# Autodesk Inventor assembly: Elo_sup
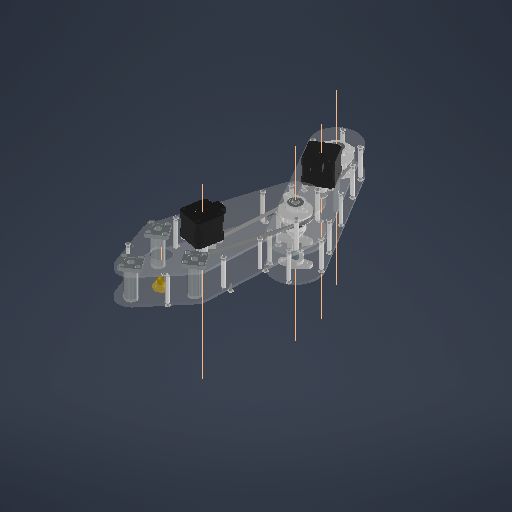
[picture p0: Inventor's stored thumbnail of the model, 512x512]
Saved by Autodesk Inventor 2025.2 (Build 292293000, 293)
## iProperties
Created: 2025-04-19
Part Number: Elo_sup
Document SubType Name: Assembly
Designer: Nelson
Author: Nelson
## Documents named in this file (19)
- C:\Users\Tiago\Documents\Inventor\Exp. Braço v1\Elo_sup.iam
- C:\Users\Tiago\Documents\Inventor\Exp. Braço v1\Veio_D8mm_L100mm.ipt
- C:\Users\Tiago\Documents\Inventor\Exp. Braço v1\RolamentoLinear10d.ipt
- C:\Users\Tiago\Documents\Inventor\Exp. Braço v1\KFL08 - Mancal Flange oval Ø8.ipt
- C:\Users\Tiago\Documents\Inventor\Exp. Braço v1\NEMA17 42-38.ipt
- C:\Users\Tiago\Documents\Inventor\Exp. Braço v1\Porca_T8.ipt
- C:\Users\Tiago\Documents\Inventor\Exp. Braço v1\Linear_Shaft_Support_SHF8.ipt
- C:\Users\Tiago\Documents\Inventor\Exp. Braço v1\1ELO.ipt
- C:\Users\Tiago\Documents\Inventor\Exp. Braço v1\2ELO.ipt
- C:\Users\Tiago\Documents\Inventor\Exp. Braço v1\3ELO.ipt
- C:\Users\Tiago\Documents\Inventor\Exp. Braço v1\4ELO.ipt
- C:\Users\Tiago\Documents\Inventor\Exp. Braço v1\espaçador_M3_L40.ipt
- C:\Users\Tiago\Documents\Inventor\Exp. Braço v1\GT2Pulley_z60.ipt
- C:\Users\Tiago\Documents\Inventor\Exp. Braço v1\GT2Pulley_z20.ipt
- C:\Users\Tiago\Documents\Inventor\Exp. Braço v1\Elo_sup\Design Accelerator\Synchronous Belts Transmission3.iam
- C:\Users\Tiago\Documents\Inventor\Exp. Braço v1\Limit_Switch_L1.ipt
- C:\Users\Tiago\Documents\Inventor\Exp. Braço v1\Elo_sup\Design Accelerator\Synchronous Belts Transmission5.iam
- C:\Users\Tiago\Documents\Inventor\Exp. Braço v1\M3 x0.5 ALT (...).ipt
- C:\Users\Tiago\Documents\Inventor\Exp. Braço v1\Anilha_M3.ipt
## Components (146 placed, 17 different names)
1. Veio_D8mm_L100mm:1 — Mate:45, Mate:48, Mate:61, Flush:3, Mate:64, Mate:65, Mate:78, Mate:82, Flush:5, Mate:143, Rotation:3, Rotation:4
2. RolamentoLinear10d:1 — Mate:54, Mate:68, Flush:4, Mate:192, Mate:193
3. RolamentoLinear10d:2 — Mate:56, Mate:190, Mate:191
4. RolamentoLinear10d:3 — Mate:57, Mate:70, Mate:194, Mate:195
5. KFL08 - Mancal Flange oval Ø8:1 — Mate:65, Mate:71, Mate:91
6. KFL08 - Mancal Flange oval Ø8:2 — Mate:63, Mate:64, Mate:74, Mate:75
7. NEMA17 42-38:1 — Mate:98, Mate:141, Mate:144, Flush:161
8. Porca_T8:1 — Mate:66, Mate:67, Mate:76, Mate:77
9. NEMA17 42-38:2 — Mate:162, Mate:163, Mate:164, Flush:159
10. Linear_Shaft_Support_SHF8:1 — Mate:45, Mate:80, Mate:81
11. Linear_Shaft_Support_SHF8:2 — Mate:48, Mate:83, Mate:84
12. Veio_D8mm_L100mm:2 — Mate:51, Mate:53, Mate:85, Mate:86, Flush:6, Mate:149
13. KFL08 - Mancal Flange oval Ø8:3 — Mate:51, Mate:87, Mate:88
14. KFL08 - Mancal Flange oval Ø8:4 — Mate:53, Mate:89, Mate:90
15. 1ELO:1 — Mate:54, Mate:56, Mate:57, Mate:61, Flush:3, Mate:63, Mate:74, Mate:75, Mate:98, Mate:100, Mate:101, Mate:102, Mate:103, Mate:104, Mate:105, Mate:106, Mate:107, Mate:121, Mate:127, Mate:144, Mate:145, Mate:146, Flush:158, Mate:157, Insert:1, Insert:4, Insert:6, Insert:8, Insert:10, Insert:12, Insert:14, Insert:16, Insert:18, Mate:182, Mate:183, Mate:184, Mate:185, Mate:186, Mate:187, Mate:188, Mate:189, Mate:190, Mate:191, Mate:192, Mate:193, Mate:194, Mate:195
16. 2ELO:1 — Mate:66, Mate:67, Mate:68, Mate:70, Flush:4, Mate:71, Mate:76, Mate:77, Distância dos elos, Mate:91, Mate:99, Mate:120, Mate:122, Mate:123, Mate:124, Mate:125, Mate:126, Mate:128, Mate:159, Mate:160, Mate:161, Angle:1, Insert:28, Insert:30, Insert:32, Insert:74, Insert:78, Insert:80, Insert:82, Insert:84, Flush:161, Insert:93
17. 3ELO:1 — Mate:78, Distância dos elos, Mate:80, Mate:81, Mate:85, Flush:6, Mate:87, Mate:88, Mate:129, Mate:130, Mate:131, Mate:132, Mate:133, Mate:134, Mate:135, Mate:136, Mate:137, Mate:138, Mate:139, Mate:140, Rotation:4, Mate:162, Mate:163, Mate:166, Mate:173, Insert:20, Insert:22, Insert:24, Insert:26, Insert:34, Insert:36, Insert:38, Insert:40, Insert:42, Insert:44, Insert:46, Insert:48, Mate:174, Mate:175, Mate:176, Mate:177, Mate:178, Mate:179, Mate:180, Mate:181
18. 4ELO:1 — Mate:82, Flush:5, Mate:83, Mate:84, Mate:86, Mate:89, Mate:90, Mate:108, Mate:109, Mate:110, Mate:111, Mate:112, Mate:113, Mate:114, Mate:115, Mate:116, Mate:117, Mate:118, Mate:119, Angle:1, Mate:167, Flush:159, Mate:173, Insert:50, Insert:52, Insert:54, Insert:56, Insert:58, Insert:60, Insert:62, Insert:64, Insert:66, Insert:68, Insert:70, Insert:94
19. espaçador_M3_L40:1 — Mate:99, Mate:100
20. espaçador_M3_L40:2 — Mate:101, Mate:126
21. espaçador_M3_L40:3 — Mate:103, Mate:123
22. espaçador_M3_L40:4 — Mate:105, Mate:122
23. espaçador_M3_L40:5 — Mate:102, Mate:127
24. espaçador_M3_L40:6 — Mate:107, Mate:125
25. espaçador_M3_L40:7 — Mate:108, Mate:130
26. espaçador_M3_L40:8 — Mate:109, Mate:131
27. espaçador_M3_L40:9 — Mate:104, Mate:128
28. espaçador_M3_L40:10 — Mate:106, Mate:124
29. espaçador_M3_L40:11 — Mate:110, Mate:129
30. espaçador_M3_L40:12 — Mate:111, Mate:135
31. espaçador_M3_L40:13 — Mate:114, Mate:138
32. espaçador_M3_L40:14 — Mate:113, Mate:139
33. espaçador_M3_L40:15 — Mate:112, Mate:140
34. espaçador_M3_L40:16 — Mate:115, Mate:136
35. espaçador_M3_L40:17 — Mate:116, Mate:137
36. espaçador_M3_L40:18 — Mate:117, Mate:134
37. espaçador_M3_L40:20 — Mate:119, Mate:132
38. espaçador_M3_L40:21 — Mate:120, Mate:121
39. espaçador_M3_L40:22 — Mate:118, Mate:133
40. GT2Pulley_z60:1 — Mate:143, Mate:145, Mate:148, Flush:7, Rotation:1, Rotation:3
41. GT2Pulley_z20:1 — Mate:141, Mate:146, Mate:147, Rotation:1
42. Synchronous Belts Transmission:3 [sub-assembly] — Mate:147, Mate:148, Flush:7
43. GT2Pulley_z20:2 — Rotation:2, Mate:164, Mate:167, Mate:169
44. GT2Pulley_z60:2 — Mate:149, Rotation:2, Mate:166, Mate:168, Flush:160
45. Limit_Switch_L1:1 — Mate:159, Mate:160, Mate:161
46. Synchronous Belts Transmission:4 [sub-assembly] — Mate:168, Mate:169, Flush:160
47. M3 x0.5 ALT (...):1 — Insert:2
48. Anilha_M3:1 — Insert:1, Insert:2
49. M3 x0.5 ALT (...):2
50. Anilha_M3:2 — Insert:4
51. M3 x0.5 ALT (...):3
52. Anilha_M3:3 — Insert:6
53. M3 x0.5 ALT (...):4
54. Anilha_M3:4 — Insert:8
55. M3 x0.5 ALT (...):5
56. Anilha_M3:5 — Insert:10
57. M3 x0.5 ALT (...):6
58. Anilha_M3:6 — Insert:12
59. M3 x0.5 ALT (...):7
60. Anilha_M3:7 — Insert:14
61. M3 x0.5 ALT (...):8
62. Anilha_M3:8 — Insert:16
63. M3 x0.5 ALT (...):9
64. Anilha_M3:9 — Insert:18
65. M3 x0.5 ALT (...):10
66. Anilha_M3:10 — Insert:20
67. M3 x0.5 ALT (...):11
68. Anilha_M3:11 — Insert:22
69. M3 x0.5 ALT (...):12
70. Anilha_M3:12 — Insert:24
71. M3 x0.5 ALT (...):13
72. Anilha_M3:13 — Insert:26
73. M3 x0.5 ALT (...):14
74. Anilha_M3:14 — Insert:28
75. M3 x0.5 ALT (...):15
76. Anilha_M3:15 — Insert:30
77. M3 x0.5 ALT (...):16
78. Anilha_M3:16 — Insert:32
79. M3 x0.5 ALT (...):17
80. Anilha_M3:17 — Insert:34
81. M3 x0.5 ALT (...):18
82. Anilha_M3:18 — Insert:36
83. M3 x0.5 ALT (...):19
84. Anilha_M3:19 — Insert:38
85. M3 x0.5 ALT (...):20
86. Anilha_M3:20 — Insert:40
87. M3 x0.5 ALT (...):21
88. Anilha_M3:21 — Insert:42
89. M3 x0.5 ALT (...):22
90. Anilha_M3:22 — Insert:44
91. M3 x0.5 ALT (...):23
92. Anilha_M3:23 — Insert:46
93. M3 x0.5 ALT (...):24
94. Anilha_M3:24 — Insert:48
95. M3 x0.5 ALT (...):25
96. Anilha_M3:25 — Insert:50
97. M3 x0.5 ALT (...):26
98. Anilha_M3:26 — Insert:52
99. M3 x0.5 ALT (...):27
100. Anilha_M3:27 — Insert:54
101. M3 x0.5 ALT (...):28
102. Anilha_M3:28 — Insert:56
103. M3 x0.5 ALT (...):29
104. Anilha_M3:29 — Insert:58
105. M3 x0.5 ALT (...):30
106. Anilha_M3:30 — Insert:60
107. M3 x0.5 ALT (...):31
108. Anilha_M3:31 — Insert:62
109. M3 x0.5 ALT (...):32
110. Anilha_M3:32 — Insert:64
111. M3 x0.5 ALT (...):33
112. Anilha_M3:33 — Insert:66
113. M3 x0.5 ALT (...):34
114. Anilha_M3:34 — Insert:68
115. M3 x0.5 ALT (...):35
116. Anilha_M3:35 — Insert:70
117. M3 x0.5 ALT (...):36
118. Anilha_M3:36 — Insert:94
119. M3 x0.5 ALT (...):37
120. Anilha_M3:37 — Insert:74
121. M3 x0.5 ALT (...):38
122. Anilha_M3:38 — Insert:93
123. M3 x0.5 ALT (...):39
124. Anilha_M3:39 — Insert:78
125. M3 x0.5 ALT (...):40
126. Anilha_M3:40 — Insert:80
127. M3 x0.5 ALT (...):41
128. Anilha_M3:41 — Insert:82
129. M3 x0.5 ALT (...):42
130. Anilha_M3:42 — Insert:84
131. M3 x0.5 ALT (...):43 — Mate:174
132. Anilha_M3:43 — Mate:175
133. M3 x0.5 ALT (...):44 — Mate:176
134. Anilha_M3:44 — Mate:177
135. M3 x0.5 ALT (...):45 — Mate:178
136. Anilha_M3:45 — Mate:181
137. M3 x0.5 ALT (...):46 — Mate:179
138. Anilha_M3:46 — Mate:180
139. M3 x0.5 ALT (...):47 — Mate:182
140. Anilha_M3:47 — Mate:187
141. M3 x0.5 ALT (...):48 — Mate:183
142. Anilha_M3:48 — Mate:189
143. M3 x0.5 ALT (...):49 — Mate:184
144. Anilha_M3:49 — Mate:186
145. M3 x0.5 ALT (...):50 — Mate:185
146. Anilha_M3:50 — Mate:188
## Relationships (226: Mate 119, Insert 92, Flush 10, RelateRotation 4, Angle 1)
- Flush:2 (-10 mm)
- Mate:45: Veio_D8mm_L100mm:1 ↔ Linear_Shaft_Support_SHF8:1
- Mate:48: Veio_D8mm_L100mm:1 ↔ Linear_Shaft_Support_SHF8:2
- Mate:51: Veio_D8mm_L100mm:2 ↔ KFL08 - Mancal Flange oval Ø8:3
- Mate:53: Veio_D8mm_L100mm:2 ↔ KFL08 - Mancal Flange oval Ø8:4
- Mate:54: RolamentoLinear10d:1 ↔ 1ELO:1
- Mate:56: RolamentoLinear10d:2 ↔ 1ELO:1
- Mate:57: RolamentoLinear10d:3 ↔ 1ELO:1
- Mate:61: Veio_D8mm_L100mm:1 ↔ 1ELO:1
- Flush:3 (-1 mm): Veio_D8mm_L100mm:1 ↔ 1ELO:1
- Mate:63: KFL08 - Mancal Flange oval Ø8:2 ↔ 1ELO:1
- Mate:64: Veio_D8mm_L100mm:1 ↔ KFL08 - Mancal Flange oval Ø8:2
- Mate:65: Veio_D8mm_L100mm:1 ↔ KFL08 - Mancal Flange oval Ø8:1
- Mate:66: Porca_T8:1 ↔ 2ELO:1
- Mate:67: Porca_T8:1 ↔ 2ELO:1
- Mate:68: RolamentoLinear10d:1 ↔ 2ELO:1
- Mate:70: RolamentoLinear10d:3 ↔ 2ELO:1
- Flush:4 (-1 mm): RolamentoLinear10d:1 ↔ 2ELO:1
- Mate:71: KFL08 - Mancal Flange oval Ø8:1 ↔ 2ELO:1
- Mate:74: KFL08 - Mancal Flange oval Ø8:2 ↔ 1ELO:1
- Mate:75: KFL08 - Mancal Flange oval Ø8:2 ↔ 1ELO:1
- Mate:76: Porca_T8:1 ↔ 2ELO:1
- Mate:77: Porca_T8:1 ↔ 2ELO:1
- Mate:78: Veio_D8mm_L100mm:1 ↔ 3ELO:1
- Distância dos elos [Mate] (6 mm): 2ELO:1 ↔ 3ELO:1
- Mate:80: Linear_Shaft_Support_SHF8:1 ↔ 3ELO:1
- Mate:81: Linear_Shaft_Support_SHF8:1 ↔ 3ELO:1
- Mate:82: Veio_D8mm_L100mm:1 ↔ 4ELO:1
- Flush:5: Veio_D8mm_L100mm:1 ↔ 4ELO:1
- Mate:83: Linear_Shaft_Support_SHF8:2 ↔ 4ELO:1
- Mate:84: Linear_Shaft_Support_SHF8:2 ↔ 4ELO:1
- Mate:85: Veio_D8mm_L100mm:2 ↔ 3ELO:1
- Mate:86: Veio_D8mm_L100mm:2 ↔ 4ELO:1
- Flush:6: Veio_D8mm_L100mm:2 ↔ 3ELO:1
- Mate:87: KFL08 - Mancal Flange oval Ø8:3 ↔ 3ELO:1
- Mate:88: KFL08 - Mancal Flange oval Ø8:3 ↔ 3ELO:1
- Mate:89: KFL08 - Mancal Flange oval Ø8:4 ↔ 4ELO:1
- Mate:90: KFL08 - Mancal Flange oval Ø8:4 ↔ 4ELO:1
- Mate:91: KFL08 - Mancal Flange oval Ø8:1 ↔ 2ELO:1
- Mate:98: NEMA17 42-38:1 ↔ 1ELO:1
- Mate:99: 2ELO:1 ↔ espaçador_M3_L40:1
- Mate:100: 1ELO:1 ↔ espaçador_M3_L40:1
- Mate:101: 1ELO:1 ↔ espaçador_M3_L40:2
- Mate:102: 1ELO:1 ↔ espaçador_M3_L40:5
- Mate:103: 1ELO:1 ↔ espaçador_M3_L40:3
- Mate:104: 1ELO:1 ↔ espaçador_M3_L40:9
- Mate:105: 1ELO:1 ↔ espaçador_M3_L40:4
- Mate:106: 1ELO:1 ↔ espaçador_M3_L40:10
- Mate:107: 1ELO:1 ↔ espaçador_M3_L40:6
- Mate:108: 4ELO:1 ↔ espaçador_M3_L40:7
- Mate:109: 4ELO:1 ↔ espaçador_M3_L40:8
- Mate:110: 4ELO:1 ↔ espaçador_M3_L40:11
- Mate:111: 4ELO:1 ↔ espaçador_M3_L40:12
- Mate:112: 4ELO:1 ↔ espaçador_M3_L40:15
- Mate:113: 4ELO:1 ↔ espaçador_M3_L40:14
- Mate:114: 4ELO:1 ↔ espaçador_M3_L40:13
- Mate:115: 4ELO:1 ↔ espaçador_M3_L40:16
- Mate:116: 4ELO:1 ↔ espaçador_M3_L40:17
- Mate:117: 4ELO:1 ↔ espaçador_M3_L40:18
- Mate:118: 4ELO:1 ↔ espaçador_M3_L40:22
- Mate:119: 4ELO:1 ↔ espaçador_M3_L40:20
- Mate:120: 2ELO:1 ↔ espaçador_M3_L40:21
- Mate:121: 1ELO:1 ↔ espaçador_M3_L40:21
- Mate:122: 2ELO:1 ↔ espaçador_M3_L40:4
- Mate:123: 2ELO:1 ↔ espaçador_M3_L40:3
- Mate:124: 2ELO:1 ↔ espaçador_M3_L40:10
- Mate:125: 2ELO:1 ↔ espaçador_M3_L40:6
- Mate:126: 2ELO:1 ↔ espaçador_M3_L40:2
- Mate:127: 1ELO:1 ↔ espaçador_M3_L40:5
- Mate:128: 2ELO:1 ↔ espaçador_M3_L40:9
- Mate:129: 3ELO:1 ↔ espaçador_M3_L40:11
- Mate:130: 3ELO:1 ↔ espaçador_M3_L40:7
- Mate:131: 3ELO:1 ↔ espaçador_M3_L40:8
- Mate:132: 3ELO:1 ↔ espaçador_M3_L40:20
- Mate:133: 3ELO:1 ↔ espaçador_M3_L40:22
- Mate:134: 3ELO:1 ↔ espaçador_M3_L40:18
- Mate:135: 3ELO:1 ↔ espaçador_M3_L40:12
- Mate:136: 3ELO:1 ↔ espaçador_M3_L40:16
- Mate:137: 3ELO:1 ↔ espaçador_M3_L40:17
- Mate:138: 3ELO:1 ↔ espaçador_M3_L40:13
- Mate:139: 3ELO:1 ↔ espaçador_M3_L40:14
- Mate:140: 3ELO:1 ↔ espaçador_M3_L40:15
- Mate:141: NEMA17 42-38:1 ↔ GT2Pulley_z20:1
- Mate:143: Veio_D8mm_L100mm:1 ↔ GT2Pulley_z60:1
- Mate:144: NEMA17 42-38:1 ↔ 1ELO:1
- Mate:145 (12 mm): 1ELO:1 ↔ GT2Pulley_z60:1
- Mate:146 (6.6 mm): 1ELO:1 ↔ GT2Pulley_z20:1
- Mate:147: GT2Pulley_z20:1 ↔ Synchronous Belts Transmission:3
- Mate:148: GT2Pulley_z60:1 ↔ Synchronous Belts Transmission:3
- Flush:7 (2.5 mm): GT2Pulley_z60:1 ↔ Synchronous Belts Transmission:3
- Rotation:1 [RelateRotation] (3 ul): GT2Pulley_z60:1 ↔ GT2Pulley_z20:1
- Mate:149: Veio_D8mm_L100mm:2 ↔ GT2Pulley_z60:2
- Rotation:2 [RelateRotation] (3 ul): GT2Pulley_z20:2 ↔ GT2Pulley_z60:2
- Flush:158: 1ELO:1
- Mate:157: 1ELO:1
- Rotation:3 [RelateRotation] (1 ul): Veio_D8mm_L100mm:1 ↔ GT2Pulley_z60:1
- Rotation:4 [RelateRotation] (1 ul): Veio_D8mm_L100mm:1 ↔ 3ELO:1
- Mate:159: 2ELO:1 ↔ Limit_Switch_L1:1
- Mate:160: 2ELO:1 ↔ Limit_Switch_L1:1
- Mate:161: 2ELO:1 ↔ Limit_Switch_L1:1
- Angle:1 (135 deg): 2ELO:1 ↔ 4ELO:1
- Mate:162: NEMA17 42-38:2 ↔ 3ELO:1
- Mate:163: NEMA17 42-38:2 ↔ 3ELO:1
- Mate:164: NEMA17 42-38:2 ↔ GT2Pulley_z20:2
- Mate:166 (12 mm): 3ELO:1 ↔ GT2Pulley_z60:2
- Mate:167 (17.6 mm): 4ELO:1 ↔ GT2Pulley_z20:2
- Flush:159 (141.105 mm): NEMA17 42-38:2 ↔ 4ELO:1
- Mate:168: GT2Pulley_z60:2 ↔ Synchronous Belts Transmission:4
- Mate:169: GT2Pulley_z20:2 ↔ Synchronous Belts Transmission:4
- Flush:160 (-2.2 mm): GT2Pulley_z60:2 ↔ Synchronous Belts Transmission:4
- Insert:1: 1ELO:1 ↔ Anilha_M3:1
- Insert:2: M3 x0.5 ALT (...):1 ↔ Anilha_M3:1
- [Insert]: M3 x0.5 ALT (...):2 ↔ Anilha_M3:2
- Insert:4: 1ELO:1 ↔ Anilha_M3:2
- [Insert]: M3 x0.5 ALT (...):3 ↔ Anilha_M3:3
- Insert:6: 1ELO:1 ↔ Anilha_M3:3
- [Insert]: M3 x0.5 ALT (...):4 ↔ Anilha_M3:4
- Insert:8: 1ELO:1 ↔ Anilha_M3:4
- [Insert]: M3 x0.5 ALT (...):5 ↔ Anilha_M3:5
- Insert:10: 1ELO:1 ↔ Anilha_M3:5
- [Insert]: M3 x0.5 ALT (...):6 ↔ Anilha_M3:6
- Insert:12: 1ELO:1 ↔ Anilha_M3:6
- [Insert]: M3 x0.5 ALT (...):7 ↔ Anilha_M3:7
- Insert:14: 1ELO:1 ↔ Anilha_M3:7
- [Insert]: M3 x0.5 ALT (...):8 ↔ Anilha_M3:8
- Insert:16: 1ELO:1 ↔ Anilha_M3:8
- [Insert]: M3 x0.5 ALT (...):9 ↔ Anilha_M3:9
- Insert:18: 1ELO:1 ↔ Anilha_M3:9
- Mate:173 (40 mm): 3ELO:1 ↔ 4ELO:1
- [Insert]: M3 x0.5 ALT (...):10 ↔ Anilha_M3:10
- Insert:20: 3ELO:1 ↔ Anilha_M3:10
- [Insert]: M3 x0.5 ALT (...):11 ↔ Anilha_M3:11
- Insert:22: 3ELO:1 ↔ Anilha_M3:11
- [Insert]: M3 x0.5 ALT (...):12 ↔ Anilha_M3:12
- Insert:24: 3ELO:1 ↔ Anilha_M3:12
- [Insert]: M3 x0.5 ALT (...):13 ↔ Anilha_M3:13
- Insert:26: 3ELO:1 ↔ Anilha_M3:13
- [Insert]: M3 x0.5 ALT (...):14 ↔ Anilha_M3:14
- Insert:28: 2ELO:1 ↔ Anilha_M3:14
- [Insert]: M3 x0.5 ALT (...):15 ↔ Anilha_M3:15
- Insert:30: 2ELO:1 ↔ Anilha_M3:15
- [Insert]: M3 x0.5 ALT (...):16 ↔ Anilha_M3:16
- Insert:32: 2ELO:1 ↔ Anilha_M3:16
- [Insert]: M3 x0.5 ALT (...):17 ↔ Anilha_M3:17
- Insert:34: 3ELO:1 ↔ Anilha_M3:17
- [Insert]: M3 x0.5 ALT (...):18 ↔ Anilha_M3:18
- Insert:36: 3ELO:1 ↔ Anilha_M3:18
- [Insert]: M3 x0.5 ALT (...):19 ↔ Anilha_M3:19
- Insert:38: 3ELO:1 ↔ Anilha_M3:19
- [Insert]: M3 x0.5 ALT (...):20 ↔ Anilha_M3:20
- Insert:40: 3ELO:1 ↔ Anilha_M3:20
- [Insert]: M3 x0.5 ALT (...):21 ↔ Anilha_M3:21
- Insert:42: 3ELO:1 ↔ Anilha_M3:21
- [Insert]: M3 x0.5 ALT (...):22 ↔ Anilha_M3:22
- Insert:44: 3ELO:1 ↔ Anilha_M3:22
- [Insert]: M3 x0.5 ALT (...):23 ↔ Anilha_M3:23
- Insert:46: 3ELO:1 ↔ Anilha_M3:23
- [Insert]: M3 x0.5 ALT (...):24 ↔ Anilha_M3:24
- Insert:48: 3ELO:1 ↔ Anilha_M3:24
- [Insert]: M3 x0.5 ALT (...):25 ↔ Anilha_M3:25
- Insert:50: 4ELO:1 ↔ Anilha_M3:25
- [Insert]: M3 x0.5 ALT (...):26 ↔ Anilha_M3:26
- Insert:52: 4ELO:1 ↔ Anilha_M3:26
- [Insert]: M3 x0.5 ALT (...):27 ↔ Anilha_M3:27
- Insert:54: 4ELO:1 ↔ Anilha_M3:27
- [Insert]: M3 x0.5 ALT (...):28 ↔ Anilha_M3:28
- Insert:56: 4ELO:1 ↔ Anilha_M3:28
- [Insert]: M3 x0.5 ALT (...):29 ↔ Anilha_M3:29
- Insert:58: 4ELO:1 ↔ Anilha_M3:29
- [Insert]: M3 x0.5 ALT (...):30 ↔ Anilha_M3:30
- Insert:60: 4ELO:1 ↔ Anilha_M3:30
- [Insert]: M3 x0.5 ALT (...):31 ↔ Anilha_M3:31
- Insert:62: 4ELO:1 ↔ Anilha_M3:31
- [Insert]: M3 x0.5 ALT (...):32 ↔ Anilha_M3:32
- Insert:64: 4ELO:1 ↔ Anilha_M3:32
- [Insert]: M3 x0.5 ALT (...):33 ↔ Anilha_M3:33
- Insert:66: 4ELO:1 ↔ Anilha_M3:33
- [Insert]: M3 x0.5 ALT (...):34 ↔ Anilha_M3:34
- Insert:68: 4ELO:1 ↔ Anilha_M3:34
- [Insert]: M3 x0.5 ALT (...):35 ↔ Anilha_M3:35
- Insert:70: 4ELO:1 ↔ Anilha_M3:35
- [Insert]: M3 x0.5 ALT (...):36 ↔ Anilha_M3:36
- [Insert]: M3 x0.5 ALT (...):37 ↔ Anilha_M3:37
- Insert:74: 2ELO:1 ↔ Anilha_M3:37
- [Insert]: M3 x0.5 ALT (...):38 ↔ Anilha_M3:38
- [Insert]: M3 x0.5 ALT (...):39 ↔ Anilha_M3:39
- Insert:78: 2ELO:1 ↔ Anilha_M3:39
- [Insert]: M3 x0.5 ALT (...):40 ↔ Anilha_M3:40
- Insert:80: 2ELO:1 ↔ Anilha_M3:40
- [Insert]: M3 x0.5 ALT (...):41 ↔ Anilha_M3:41
- Insert:82: 2ELO:1 ↔ Anilha_M3:41
- [Insert]: M3 x0.5 ALT (...):42 ↔ Anilha_M3:42
- Insert:84: 2ELO:1 ↔ Anilha_M3:42
- Flush:161 (109.63 mm): NEMA17 42-38:1 ↔ 2ELO:1
- [Insert]: M3 x0.5 ALT (...):43 ↔ Anilha_M3:43
- Mate:174: 3ELO:1 ↔ M3 x0.5 ALT (...):43
- Mate:175: 3ELO:1 ↔ Anilha_M3:43
- [Insert]: M3 x0.5 ALT (...):44 ↔ Anilha_M3:44
- Mate:176: 3ELO:1 ↔ M3 x0.5 ALT (...):44
- Mate:177: 3ELO:1 ↔ Anilha_M3:44
- [Insert]: M3 x0.5 ALT (...):45 ↔ Anilha_M3:45
- Mate:178: 3ELO:1 ↔ M3 x0.5 ALT (...):45
- [Insert]: M3 x0.5 ALT (...):46 ↔ Anilha_M3:46
- Mate:179: 3ELO:1 ↔ M3 x0.5 ALT (...):46
- Mate:180: 3ELO:1 ↔ Anilha_M3:46
- Mate:181: 3ELO:1 ↔ Anilha_M3:45
- [Insert]: M3 x0.5 ALT (...):47 ↔ Anilha_M3:47
- Mate:182: 1ELO:1 ↔ M3 x0.5 ALT (...):47
- [Insert]: M3 x0.5 ALT (...):48 ↔ Anilha_M3:48
- Mate:183: 1ELO:1 ↔ M3 x0.5 ALT (...):48
- [Insert]: M3 x0.5 ALT (...):49 ↔ Anilha_M3:49
- Mate:184: 1ELO:1 ↔ M3 x0.5 ALT (...):49
- [Insert]: M3 x0.5 ALT (...):50 ↔ Anilha_M3:50
- Mate:185: 1ELO:1 ↔ M3 x0.5 ALT (...):50
- Mate:186: 1ELO:1 ↔ Anilha_M3:49
- Mate:187: 1ELO:1 ↔ Anilha_M3:47
- Mate:188: 1ELO:1 ↔ Anilha_M3:50
- Mate:189: 1ELO:1 ↔ Anilha_M3:48
- Insert:93: 2ELO:1 ↔ Anilha_M3:38
- Insert:94: 4ELO:1 ↔ Anilha_M3:36
- Mate:190: RolamentoLinear10d:2 ↔ 1ELO:1
- Mate:191: RolamentoLinear10d:2 ↔ 1ELO:1
- Mate:192: RolamentoLinear10d:1 ↔ 1ELO:1
- Mate:193: RolamentoLinear10d:1 ↔ 1ELO:1
- Mate:194: RolamentoLinear10d:3 ↔ 1ELO:1
- Mate:195: RolamentoLinear10d:3 ↔ 1ELO:1
## Named parameters: d229_d228 = 0 mm, d231_d228 = 0 mm, d233_d228 = 0 mm, d235_d228 = 0 mm, d237_d228 = 0 mm, d239_d228 = 0 mm, d241_d228 = 0 mm, d243_d228 = 0 mm, d246_d228 = 0 mm, d248_d228 = 0 mm, d250_d228 = 0 mm, d252_d228 = 0 mm, d254_d228 = 0 mm, d256_d228 = 0 mm, d258_d228 = 0 mm, d260_d228 = 0 mm, d262_d228 = 0 mm, d264_d228 = 0 mm, d266_d228 = 0 mm, d268_d228 = 0 mm, d270_d228 = 0 mm, d272_d228 = 0 mm, d274_d228 = 0 mm, d276_d228 = 0 mm, d278_d228 = 0 mm, d280_d228 = 0 mm, d282_d228 = 0 mm, d284_d228 = 0 mm, d286_d228 = 0 mm, d288_d228 = 0 mm, d290_d228 = 0 mm, d292_d228 = 0 mm, d294_d228 = 0 mm, d296_d228 = 0 mm, d298_d228 = 0 mm, d300_d228 = 0 mm, d302_d228 = 0 mm, d304_d228 = 0 mm, d306_d228 = 0 mm, d308_d228 = 0 mm, d310_d228 = 0 mm, d315_d298_d228 = 0 mm, d318_d298_d228 = 0 mm, d321_d298_d228 = 0 mm, d323_d298_d228 = 0 mm, d327_d298_d228 = 0 mm, d329_d298_d228 = 0 mm, d331_d298_d228 = 0 mm, d333_d298_d228 = 0 mm
